# Autodesk Inventor assembly: Cheb. korp
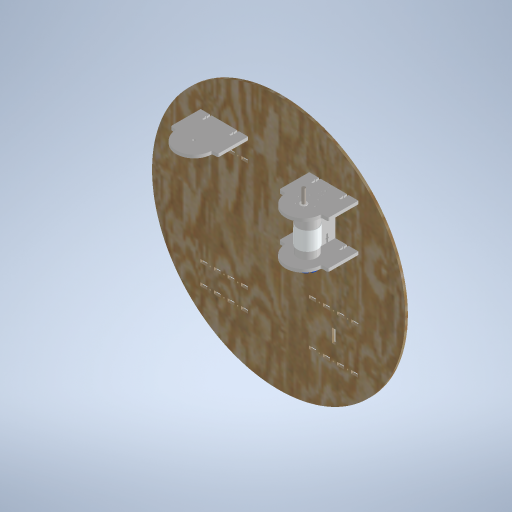
[picture p0: Inventor's stored thumbnail of the model, 512x512]
Saved by Autodesk Inventor 2023.1 (Build 271208000, 208)
## iProperties
Created: 2023-03-13
Part Number: Cheb. korp
Document SubType Name: Assembly
Designer: User
Author: User
## Documents named in this file (7)
- C:\Users\DELL\Desktop\Cheburashka_construction\Cheburashka\korpus\Cheb. korp.iam
- C:\Users\DELL\Desktop\Cheburashka_construction\Cheburashka\korpus\Osn. platform.ipt
- C:\Users\DELL\Desktop\Cheburashka_construction\Cheburashka\korpus\motor1.ipt
- C:\Users\DELL\Desktop\Cheburashka_construction\Cheburashka\korpus\motor2.ipt
- C:\Users\DELL\Desktop\Cheburashka_construction\Cheburashka\korpus\motor3.ipt
- C:\Users\DELL\Desktop\Cheburashka_construction\Cheburashka\korpus\wheel1.ipt
- C:\Users\DELL\Desktop\Cheburashka_construction\Cheburashka\korpus\Импорт\44260_txm torquenado dc motor_MIR2.ipt
## Components (6 placed, 6 different names)
1. Osn. platform:1 — Совмещение:1, Совмещение:2, Совмещение:3, Совмещение:4, Совмещение:5, Совмещение:6, Совмещение:7, Совмещение:8, Совмещение:9, Совмещение:10, Совмещение:13, Совмещение:14, Совмещение:15
2. motor1:1 — Совмещение:2, Совмещение:3, Совмещение:4
3. motor2:1 — Совмещение:5, Совмещение:6, Совмещение:7
4. motor3:1 — Совмещение:8, Совмещение:9, Совмещение:10, Совмещение:11, Совмещение:12
5. 44260_txm torquenado dc motor_MIR2:1 — Совмещение:11, Совмещение:12
6. wheel1:1 — Совмещение:13, Совмещение:14, Совмещение:15
## Relationships (15: Mate 15)
- Совмещение:1 [Mate]: Osn. platform:1
- Совмещение:2 [Mate]: Osn. platform:1 ↔ motor1:1
- Совмещение:3 [Mate]: Osn. platform:1 ↔ motor1:1
- Совмещение:4 [Mate]: Osn. platform:1 ↔ motor1:1
- Совмещение:5 [Mate]: Osn. platform:1 ↔ motor2:1
- Совмещение:6 [Mate]: Osn. platform:1 ↔ motor2:1
- Совмещение:7 [Mate]: Osn. platform:1 ↔ motor2:1
- Совмещение:8 [Mate]: Osn. platform:1 ↔ motor3:1
- Совмещение:9 [Mate]: Osn. platform:1 ↔ motor3:1
- Совмещение:10 [Mate]: Osn. platform:1 ↔ motor3:1
- Совмещение:11 [Mate]: motor3:1 ↔ 44260_txm torquenado dc motor_MIR2:1
- Совмещение:12 [Mate]: motor3:1 ↔ 44260_txm torquenado dc motor_MIR2:1
- Совмещение:13 [Mate]: Osn. platform:1 ↔ wheel1:1
- Совмещение:14 [Mate]: Osn. platform:1 ↔ wheel1:1
- Совмещение:15 [Mate]: Osn. platform:1 ↔ wheel1:1
